# Autodesk Inventor assembly: Version1
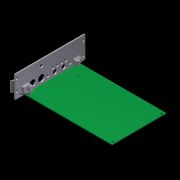
[picture p0: Inventor's stored thumbnail of the model, 180x180]
Saved by Autodesk Inventor 2011 SP1 (Build 150282100, 282)
## iProperties
Created: 2012-07-18
Part Number: Version1
Document SubType Name: Assembly
Designer: nfischer
Author: nfischer
## Documents named in this file (7)
- D:\Programmieren\C-Programmieren\Frontplatte\Version1.iam
- D:\Programmieren\C-Programmieren\Frontplatte\Grundsätzliches\0.5_Lochrasterplatine.ipt
- D:\Programmieren\C-Programmieren\Frontplatte\Grundsätzliches\0.1_Lagerbuchse.ipt
- D:\Programmieren\C-Programmieren\Frontplatte\Grundsätzliches\0.2_Frontgriff.ipt
- D:\Programmieren\C-Programmieren\Frontplatte\Grundsätzliches\0.3_Leiterplattenhalter_Links.ipt
- D:\Programmieren\C-Programmieren\Frontplatte\Grundsätzliches\0.4_Leiterplattenhalter_Rechts.ipt
- D:\Programmieren\C-Programmieren\Frontplatte\Grundsätzliches\FrontplatteFG698.ipt
## Components (6 placed, 6 different names)
1. 0.5_Lochrasterplatine:1 — Einfügen:3, Einfügen:5
2. 0.1_Lagerbuchse:1 — Einfügen:3, Einfügen:4, Passend:1
3. 0.2_Frontgriff:1 — Einfügen:4, Winkel:3
4. 0.3_Leiterplattenhalter_Links:1 — Einfügen:1, Winkel:2, Einfügen:5
5. 0.4_Leiterplattenhalter_Rechts:1 — Einfügen:2, Winkel:1, Passend:1
6. FrontplatteFG698:1 — Einfügen:1, Einfügen:2, Winkel:1, Winkel:2, Winkel:3
## Relationships (9: Insert 5, Angle 3, Mate 1)
- Einfügen:1 [Insert]: 0.3_Leiterplattenhalter_Links:1 ↔ FrontplatteFG698:1
- Einfügen:2 [Insert]: 0.4_Leiterplattenhalter_Rechts:1 ↔ FrontplatteFG698:1
- Einfügen:3 [Insert]: 0.5_Lochrasterplatine:1 ↔ 0.1_Lagerbuchse:1
- Einfügen:4 [Insert]: 0.1_Lagerbuchse:1 ↔ 0.2_Frontgriff:1
- Winkel:1 [Angle] (0 deg): 0.4_Leiterplattenhalter_Rechts:1 ↔ FrontplatteFG698:1
- Winkel:2 [Angle] (0 deg): 0.3_Leiterplattenhalter_Links:1 ↔ FrontplatteFG698:1
- Einfügen:5 [Insert]: 0.5_Lochrasterplatine:1 ↔ 0.3_Leiterplattenhalter_Links:1
- Passend:1 [Mate]: 0.1_Lagerbuchse:1 ↔ 0.4_Leiterplattenhalter_Rechts:1
- Winkel:3 [Angle] (0 deg): 0.2_Frontgriff:1 ↔ FrontplatteFG698:1
